# Autodesk Inventor assembly: Arm Assembly
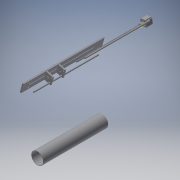
[picture p0: Inventor's stored thumbnail of the model, 180x180]
Saved by Autodesk Inventor 2016 (Build 200138000, 138)
## iProperties
Created: 2016-04-23
Part Number: Arm Assembly
Document SubType Name: Assembly
Designer: rubenjm
Author: rubenjm
## Documents named in this file (9)
- C:\Users\rubenjm\Documents\To Transfer\2k16 Spring\RME\GGC\V3\Arm Assembly.iam
- C:\Users\rubenjm\Documents\To Transfer\2k16 Spring\RME\GGC\V3\Inner Pole.ipt
- C:\Users\rubenjm\Documents\To Transfer\2k16 Spring\RME\GGC\V3\Arm Base.ipt
- C:\Users\rubenjm\Documents\To Transfer\2k16 Spring\RME\GGC\V3\Holder.ipt
- C:\Users\rubenjm\Documents\To Transfer\2k16 Spring\RME\GGC\V3\Threaded Rod Nut.ipt
- C:\Users\rubenjm\Documents\To Transfer\2k16 Spring\RME\GGC\V3\Unthreaded Rod.ipt
- C:\Users\rubenjm\Documents\To Transfer\2k16 Spring\RME\GGC\V3\Threaded Rod.ipt
- C:\Users\rubenjm\Documents\To Transfer\2k16 Spring\RME\GGC\V3\NEMA23 Motor.ipt
- C:\Users\rubenjm\Documents\To Transfer\2k16 Spring\RME\GGC\V3\Motor Coupler.ipt
## Components (11 placed, 8 different names)
1. Inner Pole:1
2. Arm Base:1 — Mate:1, Mate:2, Mate:15
3. Holder:1 — Mate:1, Mate:2, Mate:8, Mate:9, Mate:10, Mate:12, Mate:13, Mate:21
4. Holder:2 — Mate:15, Mate:16, Mate:17, Mate:18, Mate:19, Mate:20, Mate:21
5. Threaded Rod Nut:1 — Mate:8, Mate:9, Mate:10, Mate:11
6. Threaded Rod Nut:2 — Mate:18, Mate:19, Mate:20
7. Unthreaded Rod:1 — Mate:13, Mate:16
8. Unthreaded Rod:2 — Mate:12, Mate:17
9. Threaded Rod:1 — Mate:11, Mate:24, Mate:25
10. NEMA23 Motor:1 — Mate:22, Mate:23
11. Motor Coupler:1 — Mate:22, Mate:23, Mate:24, Mate:25
## Relationships (19: Mate 19)
- Mate:1: Arm Base:1 ↔ Holder:1
- Mate:2: Arm Base:1 ↔ Holder:1
- Mate:8: Holder:1 ↔ Threaded Rod Nut:1
- Mate:9: Holder:1 ↔ Threaded Rod Nut:1
- Mate:10: Holder:1 ↔ Threaded Rod Nut:1
- Mate:11: Threaded Rod Nut:1 ↔ Threaded Rod:1
- Mate:12: Holder:1 ↔ Unthreaded Rod:2
- Mate:13: Holder:1 ↔ Unthreaded Rod:1
- Mate:15: Arm Base:1 ↔ Holder:2
- Mate:16: Holder:2 ↔ Unthreaded Rod:1
- Mate:17: Holder:2 ↔ Unthreaded Rod:2
- Mate:18: Holder:2 ↔ Threaded Rod Nut:2
- Mate:19: Holder:2 ↔ Threaded Rod Nut:2
- Mate:20: Holder:2 ↔ Threaded Rod Nut:2
- Mate:21 (101.6 mm): Holder:1 ↔ Holder:2
- Mate:22: NEMA23 Motor:1 ↔ Motor Coupler:1
- Mate:23: NEMA23 Motor:1 ↔ Motor Coupler:1
- Mate:24: Threaded Rod:1 ↔ Motor Coupler:1
- Mate:25: Threaded Rod:1 ↔ Motor Coupler:1
